# Autodesk Inventor assembly: prototype7
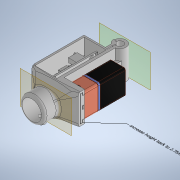
[picture p0: Inventor's stored thumbnail of the model, 180x180]
Saved by Autodesk Inventor 2022 (Build 260153000, 153)
## iProperties
Created: 2022-06-15
Part Number: prototype7
Document SubType Name: Assembly
Designer: tecware
Author: tecware
## Documents named in this file (6)
- C:\Users\tecware\Documents\git\calibrationKit\calibrationKit_v2\wand\prototype_for_circuit&connections\prototype_12.iam
- C:\Users\tecware\Documents\git\calibrationKit\calibrationKit_v2\wand\prototype_for_circuit&connections\prototype_11_2.ipt
- C:\Users\tecware\Documents\git\calibrationKit\calibrationKit_v2\wand\prototype_for_circuit&connections\prototype_12_1.ipt
- C:\Users\tecware\Documents\git\calibrationKit\calibrationKit_v2\wand\prototype_for_circuit&connections\prototype_12_cover.ipt
- C:\Users\tecware\Documents\git\calibrationKit\calibrationKit_v2\components\Buck Boost Converter\_xl6009_dc-dc_boost_buck.iam
- C:\Users\tecware\Documents\git\calibrationKit\calibrationKit_v2\components\9V Battery\9V Battery.ipt
## Components (5 placed, 5 different names)
1. prototype_12_1:1 — Flush:1, Flush:2, Mate:1, Mate:2, Mate:3, Mate:4, Mate:5, Mate:6
2. prototype_11_2:1 — Flush:1, Flush:2, Mate:1
3. prototype_12_cover:1
4. _xl6009_dc-dc_boost_buck:1 [sub-assembly] — Mate:5, Mate:6
5. 9V Battery:1 — Mate:2, Mate:3, Mate:4
## Relationships (8: Mate 6, Flush 2)
- Flush:1: prototype_12_1:1 ↔ prototype_11_2:1
- Flush:2: prototype_12_1:1 ↔ prototype_11_2:1
- Mate:1 (0.2 mm): prototype_12_1:1 ↔ prototype_11_2:1
- Mate:2: prototype_12_1:1 ↔ 9V Battery:1
- Mate:3: prototype_12_1:1 ↔ 9V Battery:1
- Mate:4: prototype_12_1:1 ↔ 9V Battery:1
- Mate:5: prototype_12_1:1 ↔ _xl6009_dc-dc_boost_buck:1
- Mate:6: prototype_12_1:1 ↔ _xl6009_dc-dc_boost_buck:1
